# Autodesk Inventor assembly: Rail_Assembly
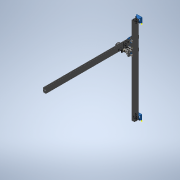
[picture p0: Inventor's stored thumbnail of the model, 180x180]
Saved by Autodesk Inventor 2021 (Build 250183000, 183)
## iProperties
Created: 2021-01-25
Part Number: Rail_Assembly
Document SubType Name: Assembly
Designer: Jorian Brusind
Mass: 3786.54 g
Surface Area: 19508.5 cm^2
Volume: 2323.9 cm^3
Density: 1.62939 g/cm^3
Author: Jorian Brusind
## Documents named in this file (18)
- C:\Users\Jorian Brusind\Documents\GitHub\PersonalProjects\HyperRail\Inventor Files\Rail_Assembly.iam
- C:\Users\Jorian Brusind\Documents\GitHub\PersonalProjects\Inventor Projects\Useful models\NEMA_Steppers\NEMA23\23HS8430B.ipt
- C:\Users\Jorian Brusind\Documents\GitHub\PersonalProjects\HyperRail\Inventor Files\NEMA23_StepperonlineMount.ipt
- C:\Users\Jorian Brusind\Documents\GitHub\PersonalProjects\HyperRail\Inventor Files\Roller_Bracket.iam
- C:\Users\Jorian Brusind\Documents\GitHub\PersonalProjects\Inventor Projects\Useful models\8020_Sets\IPT_40_Series\Extra_40_Series\HFS5-4060-4000\HFS5-4060-1275.ipt
- C:\Users\Jorian Brusind\Documents\GitHub\PersonalProjects\Inventor Projects\Useful models\8020_Sets\IPT_20_Series\IPT_20_Series\20-2040_200mm.ipt
- C:\Users\Jorian Brusind\Documents\GitHub\PersonalProjects\HyperRail\Inventor Files\2804S_NEMA2115_1Gearbox.ipt
- C:\Users\Jorian Brusind\Documents\GitHub\PersonalProjects\Inventor Projects\Useful models\8020_Sets\IPT_40_Series\Extra_40_Series\90deg_4040.ipt
- C:\Users\Jorian Brusind\Documents\GitHub\PersonalProjects\HyperRail\Inventor Files\Bottom_Stand.ipt
- C:\Users\Jorian Brusind\Documents\GitHub\PersonalProjects\HyperRail\Inventor Files\SmallBelt_LargePulley.ipt
- C:\Users\Jorian Brusind\Documents\GitHub\PersonalProjects\HyperRail\Inventor Files\11mm_BearingWheel.ipt
- C:\Users\Jorian Brusind\Documents\GitHub\PersonalProjects\Inventor Projects\Useful models\Metric bolt\Bolt M5 25mm.ipt
- C:\Users\Jorian Brusind\Documents\GitHub\PersonalProjects\HyperRail\Inventor Files\Idlepulley_Spacer.ipt
- C:\Users\Jorian Brusind\Documents\GitHub\PersonalProjects\HyperRail\Inventor Files\Small_belt_5mm_1mm.ipt
- C:\Users\Jorian Brusind\Documents\GitHub\PersonalProjects\Inventor Projects\Useful models\8020_Sets\IPT_20_Series\Extra_20_Series\8020_14056m\14056_m.ipt
- C:\Users\Jorian Brusind\Documents\GitHub\PersonalProjects\HyperRail\PCB Files\Integrated Stepper Motor Driver\ExportSTEP\Main.iam
- C:\Users\Jorian Brusind\Documents\GitHub\PersonalProjects\HyperRail\Inventor Files\NEMA23_Shroud.ipt
- C:\Users\Jorian Brusind\Documents\GitHub\PersonalProjects\HyperRail\Inventor Files\NEMA23_Shroud_Cover.ipt
## Components (25 placed, 17 different names)
1. 23HS8430B:1 — Angle:1, Mate:97, Mate:125, Flush:54, Flush:55, Mate:127, Mate:129, Mate:130
2. NEMA23_StepperonlineMount:1 — Angle:1, Angle:2, Flush:14, Mate:98, Flush:41, Mate:101, Mate:104, Mate:106, Mate:126, Mate:128
3. Roller_Bracket:1 [sub-assembly] — Flush:43, Flush:45, Mate:112, Mate:113, Flush:48, Mate:114, Mate:117, Flush:50, Mate:120, Flush:51
4. Roller_Bracket:2 [sub-assembly] — Flush:43, Flush:48, Flush:49, Mate:115, Mate:122, Flush:52, Mate:123, Flush:53
5. HFS5-4060-1275:1 — Mate:70, Flush:22, Mate:71, Mate:91, Mate:92, Mate:93, Mate:94, Mate:95, Mate:96, Mate:107, Mate:108, Mate:110, Mate:112, Mate:114, Mate:115, Mate:116
6. HFS5-4060-1275:2 — Flush:10, Mate:56, Flush:14, Mate:82, Mate:84, Flush:41, Mate:126
7. 20-2040_200mm:1 — Flush:10, Mate:56, Flush:34, Mate:83, Flush:35, Flush:36, Mate:85, Flush:45, Mate:113, Flush:49, Mate:118, Mate:119, Mate:121, Mate:124
8. 2804S_NEMA2115_1Gearbox:1 — Angle:2, Mate:97, Mate:98, Mate:99, Mate:100, Mate:109, Mate:127, Mate:128
9. 90deg_4040:1 — Mate:82, Flush:34, Mate:83, Flush:35
10. 90deg_4040:2 — Mate:84, Flush:36, Mate:85
11. Bottom_Stand:1 — Mate:91, Mate:92, Mate:93
12. Bottom_Stand:2 — Mate:94, Mate:95, Mate:96
13. SmallBelt_LargePulley:1 — Mate:99, Mate:100
14. 11mm_BearingWheel:1 — Mate:101, Mate:102, Mate:103, Mate:104
15. Bolt M5 25mm:1 — Mate:102, Mate:103, Mate:105, Mate:116
16. Idlepulley_Spacer:1 — Mate:105, Mate:106
17. Small_belt_5mm_1mm:1 — Mate:107, Mate:108, Mate:109, Flush:42, Mate:111
18. Small_belt_5mm_1mm:2 — Flush:42, Mate:110, Mate:111
19. 14056_m:1 — Mate:117, Mate:118, Flush:50
20. 14056_m:2 — Mate:119, Mate:120, Flush:51
21. 14056_m:3 — Mate:121, Mate:122, Flush:52
22. 14056_m:4 — Mate:123, Mate:124, Flush:53
23. Main:1 [sub-assembly] — Mate:125, Flush:54, Flush:55
24. NEMA23_Shroud:1 — Mate:129, Mate:130, Mate:131, Mate:132
25. NEMA23_Shroud_Cover:1 — Mate:131, Mate:132
## Relationships (69: Mate 49, Flush 18, Angle 2)
- Angle:1 (0 deg): 23HS8430B:1 ↔ NEMA23_StepperonlineMount:1
- Flush:10: HFS5-4060-1275:2 ↔ 20-2040_200mm:1
- Angle:2 (0 deg): NEMA23_StepperonlineMount:1 ↔ 2804S_NEMA2115_1Gearbox:1
- Mate:56: HFS5-4060-1275:2 ↔ 20-2040_200mm:1
- Flush:14 (-60 mm): NEMA23_StepperonlineMount:1 ↔ HFS5-4060-1275:2
- Mate:70: HFS5-4060-1275:1
- Flush:22: HFS5-4060-1275:1
- Mate:71: HFS5-4060-1275:1
- Mate:82: HFS5-4060-1275:2 ↔ 90deg_4040:1
- Flush:34: 20-2040_200mm:1 ↔ 90deg_4040:1
- Mate:83: 20-2040_200mm:1 ↔ 90deg_4040:1
- Flush:35: 20-2040_200mm:1 ↔ 90deg_4040:1
- Mate:84: HFS5-4060-1275:2 ↔ 90deg_4040:2
- Flush:36: 20-2040_200mm:1 ↔ 90deg_4040:2
- Mate:85: 20-2040_200mm:1 ↔ 90deg_4040:2
- Mate:91: HFS5-4060-1275:1 ↔ Bottom_Stand:1
- Mate:92: HFS5-4060-1275:1 ↔ Bottom_Stand:1
- Mate:93: HFS5-4060-1275:1 ↔ Bottom_Stand:1
- Mate:94: HFS5-4060-1275:1 ↔ Bottom_Stand:2
- Mate:95: HFS5-4060-1275:1 ↔ Bottom_Stand:2
- Mate:96: HFS5-4060-1275:1 ↔ Bottom_Stand:2
- Mate:97: 23HS8430B:1 ↔ 2804S_NEMA2115_1Gearbox:1
- Mate:98: NEMA23_StepperonlineMount:1 ↔ 2804S_NEMA2115_1Gearbox:1
- Flush:41 (-2 mm): NEMA23_StepperonlineMount:1 ↔ HFS5-4060-1275:2
- Mate:99: 2804S_NEMA2115_1Gearbox:1 ↔ SmallBelt_LargePulley:1
- Mate:100 (4 mm): 2804S_NEMA2115_1Gearbox:1 ↔ SmallBelt_LargePulley:1
- Mate:101: NEMA23_StepperonlineMount:1 ↔ 11mm_BearingWheel:1
- Mate:102: 11mm_BearingWheel:1 ↔ Bolt M5 25mm:1
- Mate:103: 11mm_BearingWheel:1 ↔ Bolt M5 25mm:1
- Mate:104 (10 mm): NEMA23_StepperonlineMount:1 ↔ 11mm_BearingWheel:1
- Mate:105: Bolt M5 25mm:1 ↔ Idlepulley_Spacer:1
- Mate:106: NEMA23_StepperonlineMount:1 ↔ Idlepulley_Spacer:1
- Mate:107: HFS5-4060-1275:1 ↔ Small_belt_5mm_1mm:1
- Mate:108: HFS5-4060-1275:1 ↔ Small_belt_5mm_1mm:1
- Mate:109 (10 mm): 2804S_NEMA2115_1Gearbox:1 ↔ Small_belt_5mm_1mm:1
- Flush:42: Small_belt_5mm_1mm:1 ↔ Small_belt_5mm_1mm:2
- Mate:110: HFS5-4060-1275:1 ↔ Small_belt_5mm_1mm:2
- Mate:111 (20 mm): Small_belt_5mm_1mm:1 ↔ Small_belt_5mm_1mm:2
- Flush:43: Roller_Bracket:1 ↔ Roller_Bracket:2
- Flush:45: Roller_Bracket:1 ↔ 20-2040_200mm:1
- Mate:112: Roller_Bracket:1 ↔ HFS5-4060-1275:1
- Mate:113: Roller_Bracket:1 ↔ 20-2040_200mm:1
- Flush:48: Roller_Bracket:1 ↔ Roller_Bracket:2
- Flush:49: Roller_Bracket:2 ↔ 20-2040_200mm:1
- Mate:114 (11 mm): Roller_Bracket:1 ↔ HFS5-4060-1275:1
- Mate:115 (11 mm): Roller_Bracket:2 ↔ HFS5-4060-1275:1
- Mate:116 (11 mm): HFS5-4060-1275:1 ↔ Bolt M5 25mm:1
- Mate:117: Roller_Bracket:1 ↔ 14056_m:1
- Mate:118: 20-2040_200mm:1 ↔ 14056_m:1
- Flush:50: Roller_Bracket:1 ↔ 14056_m:1
- Mate:119: 20-2040_200mm:1 ↔ 14056_m:2
- Mate:120: Roller_Bracket:1 ↔ 14056_m:2
- Flush:51: Roller_Bracket:1 ↔ 14056_m:2
- Mate:121: 20-2040_200mm:1 ↔ 14056_m:3
- Mate:122: Roller_Bracket:2 ↔ 14056_m:3
- Flush:52: Roller_Bracket:2 ↔ 14056_m:3
- Mate:123: Roller_Bracket:2 ↔ 14056_m:4
- Mate:124: 20-2040_200mm:1 ↔ 14056_m:4
- Flush:53: Roller_Bracket:2 ↔ 14056_m:4
- Mate:125 (1 mm): 23HS8430B:1 ↔ Main:1
- Flush:54 (7 mm): 23HS8430B:1 ↔ Main:1
- Flush:55 (7 mm): 23HS8430B:1 ↔ Main:1
- Mate:126: NEMA23_StepperonlineMount:1 ↔ HFS5-4060-1275:2
- Mate:127: 23HS8430B:1 ↔ 2804S_NEMA2115_1Gearbox:1
- Mate:128: NEMA23_StepperonlineMount:1 ↔ 2804S_NEMA2115_1Gearbox:1
- Mate:129: 23HS8430B:1 ↔ NEMA23_Shroud:1
- Mate:130: 23HS8430B:1 ↔ NEMA23_Shroud:1
- Mate:131: NEMA23_Shroud:1 ↔ NEMA23_Shroud_Cover:1
- Mate:132: NEMA23_Shroud:1 ↔ NEMA23_Shroud_Cover:1
